# Autodesk Inventor assembly: HexShaft+Toughbox-mini
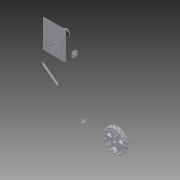
[picture p0: Inventor's stored thumbnail of the model, 180x180]
Saved by Autodesk Inventor 2013 (Build 170138000, 138)
## iProperties
Created: 2013-01-11
Part Number: HexShaft+Toughbox-mini
Document SubType Name: Assembly
Designer: Naphat
Translation Standard: STEP AP203
FileName: S:/Products/Gearboxes Spur Single Stage/Toughbox/Toughbox Mini/Toughbox-Mini.stp
PreProcessor: Unknown
PostProcessor: Build: 138, Release: 2013 RTM - Date: Thu 03/01/2012
Sent Units: millimeter
Uncertainty: 0.001
Author: Naphat
## Documents named in this file (19)
- C:\Users\carneeki\Desktop\Kiwi Robot\Drive Wheel\Drive Wheel.iam
- C:\Users\carneeki\Desktop\Kiwi Robot\Imported Components\Toughbox-mini\r6zz.ipt
- C:\Users\carneeki\Desktop\Kiwi Robot\Imported Components\Toughbox-mini\Toughbox_d07.ipt
- C:\Users\carneeki\Desktop\Kiwi Robot\Imported Components\Toughbox-mini\Toughbox_d05.ipt
- C:\Users\carneeki\Desktop\Kiwi Robot\Imported Components\Toughbox-mini\Toughbox_d08.ipt
- C:\Users\carneeki\Desktop\Kiwi Robot\Imported Components\Toughbox-mini\Toughbox_d06.ipt
- C:\Users\carneeki\Desktop\Kiwi Robot\Imported Components\Toughbox-mini\fr-6-zz.ipt
- C:\Users\carneeki\Desktop\Kiwi Robot\Imported Components\Toughbox-mini\fr-8-zz.ipt
- C:\Users\carneeki\Desktop\Kiwi Robot\Imported Components\Toughbox-mini\10-32_nylock_nut.ipt
- C:\Users\carneeki\Desktop\Kiwi Robot\Imported Components\Toughbox-mini\5-16_washer.ipt
- C:\Users\carneeki\Desktop\Kiwi Robot\Imported Components\Toughbox-mini\Toughbox_d09.ipt
- C:\Users\carneeki\Desktop\Kiwi Robot\Imported Components\Toughbox-mini\8mm_spring_clip.ipt
- C:\Users\carneeki\Desktop\Kiwi Robot\Imported Components\Toughbox-mini\Toughbox-mini_d01-5-12.ipt
- C:\Users\carneeki\Desktop\Kiwi Robot\Imported Components\Toughbox-mini\10-32x0625_shcs.ipt
- C:\Users\carneeki\Desktop\Kiwi Robot\Imported Components\Motors\CIM\CIM Motor.iam
- C:\Users\carneeki\Desktop\Kiwi Robot\Drive Wheel\CustomAM-2230.ipt
- C:\Users\carneeki\Desktop\Kiwi Robot\Imported Components\217-2613.20121203\217-2613.20121203.iam
- C:\Users\carneeki\Desktop\Kiwi Robot\Imported Components\217-2592.20121203.ipt
- C:\Users\carneeki\Desktop\Kiwi Robot\Imported Components\Hex Shaft.ipt
## Components (35 placed, 18 different names)
1. CIM Motor [sub-assembly]
2. CustomAM-2230:1 — Mate:10, Mate:11
3. 217-2613.20121203:1 [sub-assembly] — Insert:1, Insert:2, Mate:17, Mate:18
4. 217-2592.20121203:1 — Insert:2, Mate:17, Mate:18
5. 217-2592.20121203:2 — Mate:14, Mate:15, Mate:16, Insert:1
6. Hex Shaft:1 — Mate:12, Mate:13, Flush:1, Mate:14, Mate:15
7. r6zz:1
8. r6zz:2 — Mate:9
9. Toughbox_d07:1
10. Toughbox_d05:1
11. Toughbox_d08:1
12. Toughbox_d06:1 — Mate:12, Mate:13
13. fr-6-zz:1 — Mate:10
14. fr-8-zz:1 — Mate:11, Mate:16
15. 10-32_nylock_nut:1
16. 10-32_nylock_nut:2
17. 10-32_nylock_nut:3
18. 10-32_nylock_nut:4
19. 5-16_washer:1
20. 5-16_washer:2
21. 5-16_washer:3
22. 5-16_washer:4
23. Toughbox_d09:1
24. Toughbox_d09:2
25. 8mm_spring_clip:1
26. 8mm_spring_clip:2
27. Toughbox-mini_d01-5-12:1 — Mate:9, Flush:1
28. 10-32x0625_shcs:1
29. 10-32x0625_shcs:2
30. 10-32x0625_shcs:3
31. 10-32x0625_shcs:4
32. 10-32x0625_shcs:5
33. 10-32x0625_shcs:6
34. 10-32x0625_shcs:7
35. 10-32x0625_shcs:8
## Relationships (13: Mate 10, Insert 2, Flush 1)
- Mate:9: r6zz:2 ↔ Toughbox-mini_d01-5-12:1
- Mate:10: CustomAM-2230:1 ↔ fr-6-zz:1
- Mate:11: CustomAM-2230:1 ↔ fr-8-zz:1
- Mate:12: Hex Shaft:1 ↔ Toughbox_d06:1
- Mate:13: Hex Shaft:1 ↔ Toughbox_d06:1
- Flush:1: Hex Shaft:1 ↔ Toughbox-mini_d01-5-12:1
- Mate:14: 217-2592.20121203:2 ↔ Hex Shaft:1
- Mate:15: 217-2592.20121203:2 ↔ Hex Shaft:1
- Mate:16 (2 mm): 217-2592.20121203:2 ↔ fr-8-zz:1
- Insert:1: 217-2613.20121203:1 ↔ 217-2592.20121203:2
- Insert:2: 217-2613.20121203:1 ↔ 217-2592.20121203:1
- Mate:17: 217-2613.20121203:1 ↔ 217-2592.20121203:1
- Mate:18: 217-2613.20121203:1 ↔ 217-2592.20121203:1
